# Autodesk Inventor assembly: Assembly1
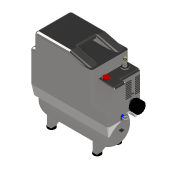
[picture p0: Inventor's stored thumbnail of the model, 180x180]
Saved by Autodesk Inventor 2019 (Build 230136000, 136)
## iProperties
Created: 2020-05-05
Part Number: Assembly1
Document SubType Name: Assembly
Designer: IVAN
Author: IVAN
## Documents named in this file (3)
- F:\IVAN\Kuliah\TA\NEW DESAIN 3D\DESAIN 3D\Compresor\Assembly1.iam
- F:\IVAN\Kuliah\TA\NEW DESAIN 3D\DESAIN 3D\Compresor\Part1.ipt
- F:\IVAN\Kuliah\TA\NEW DESAIN 3D\DESAIN 3D\Compresor\Part2.ipt
## Components (2 placed, 2 different names)
1. Part1:1 — Mate:1, Flush:2
2. Part2:1 — Flush:1, Mate:1, Flush:2
## Relationships (3: Flush 2, Mate 1)
- Flush:1 (-90 mm): Part2:1
- Mate:1: Part1:1 ↔ Part2:1
- Flush:2: Part1:1 ↔ Part2:1
